# Autodesk Inventor assembly: test_stand_cable_pose_configuration
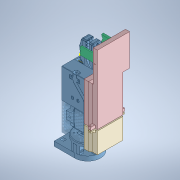
[picture p0: Inventor's stored thumbnail of the model, 180x180]
Saved by Autodesk Inventor 2022 (Build 260153000, 153)
## iProperties
Created: 2022-03-16
Part Number: test_stand_cable_pose_configuration
Document SubType Name: Assembly
Designer: kylem
Author: kylem
## Documents named in this file (5)
- C:\Users\kylem\OneDrive\Documents\GitHub\IMML_Contactile_Gripper_Hardware\test_stand\test_stand_cable_pose_configuration.iam
- C:\Users\kylem\OneDrive\Documents\GitHub\IMML_Contactile_Gripper_Hardware\Gripper_Design_NonCompliant_No_UR5.iam
- C:\Users\kylem\OneDrive\Documents\GitHub\IMML_Contactile_Gripper_Hardware\test_stand\cable_jig_base.ipt
- C:\Users\kylem\OneDrive\Documents\GitHub\IMML_Contactile_Gripper_Hardware\test_stand\cable_jig_holder_v0.ipt
- C:\Users\kylem\OneDrive\Documents\GitHub\IMML_Contactile_Gripper_Hardware\test_stand\cable_jig_base_back.ipt
## Components (4 placed, 4 different names)
1. Gripper_Design_NonCompliant_No_UR5:1 [sub-assembly] — Mate:1, Mate:2, Mate:4, Mate:5, Mate:6
2. cable_jig_base:1 — Mate:1, Mate:2, Mate:7, Mate:8
3. cable_jig_holder_v0:1 — Mate:7, Mate:8
4. cable_jig_base_back:1 — Mate:4, Mate:5, Mate:6
## Relationships (7: Mate 7)
- Mate:1: Gripper_Design_NonCompliant_No_UR5:1 ↔ cable_jig_base:1
- Mate:2 (0.125 mm): Gripper_Design_NonCompliant_No_UR5:1 ↔ cable_jig_base:1
- Mate:4: Gripper_Design_NonCompliant_No_UR5:1 ↔ cable_jig_base_back:1
- Mate:5 (0.125 mm): Gripper_Design_NonCompliant_No_UR5:1 ↔ cable_jig_base_back:1
- Mate:6: Gripper_Design_NonCompliant_No_UR5:1 ↔ cable_jig_base_back:1
- Mate:7: cable_jig_base:1 ↔ cable_jig_holder_v0:1
- Mate:8: cable_jig_base:1 ↔ cable_jig_holder_v0:1
